# Autodesk Inventor assembly: SaponseEx
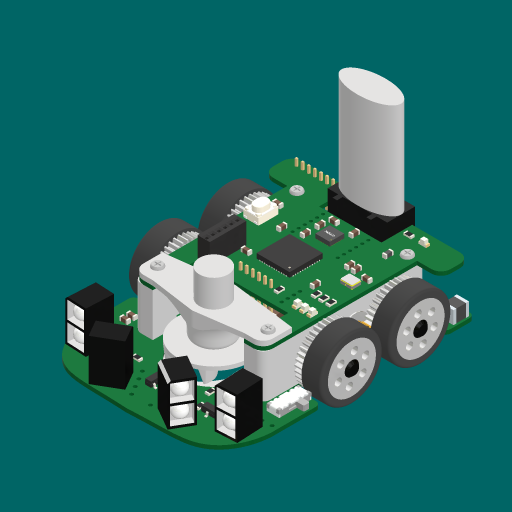
[picture p0: Inventor's stored thumbnail of the model, 512x512]
Saved by Autodesk Inventor 2023 (Build 270158000, 158)
## iProperties
Created: 2022-09-02
Part Number: SaponseEx
Document SubType Name: Assembly
Designer: neko2
Mass: 18.3356 g
Surface Area: 212.041 cm^2
Volume: 11.0257 cm^3
Density: 1.66299 g/cm^3
Author: neko2
## Documents named in this file (13)
- C:\Users\hide\Desktop\SaponseEx\CAD\SaponseEx.iam
- C:\Users\hide\Desktop\SaponseEx\CAD\足回り.iam
- C:\Users\hide\Desktop\SaponseEx\CAD\PCB\SaponseEx_PCB.ipt
- C:\Users\hide\Desktop\SaponseEx\CAD\Board_Parts\SNZS-M1_6-4.ipt
- C:\Users\hide\Desktop\SaponseEx\CAD\PCB\Brains_PCB.ipt
- C:\Users\hide\Desktop\SaponseEx\CAD\PCB\EncL_PCB.ipt
- C:\Users\hide\Desktop\SaponseEx\CAD\PCB\EncR_PCB.ipt
- C:\Users\hide\Desktop\SaponseEx\CAD\Board_Parts\Lipo.ipt
- C:\Users\hide\Desktop\SaponseEx\CAD\吸引\FanMotorMount.ipt
- C:\Users\hide\Desktop\SaponseEx\CAD\mirror\足回り_MIR.iam
- C:\Users\hide\Desktop\SaponseEx\CAD\Skirt.ipt
- C:\Users\hide\Desktop\SaponseEx\CAD\吸引\FanMotor.ipt
- C:\Users\hide\Desktop\SaponseEx\CAD\吸引\Fan4.ipt
## Components (19 placed, 12 different names)
1. SaponseEx_PCB:1 — フラッシュ:1, フラッシュ:2, メイト:1, メイト:10, メイト:11, メイト:12, メイト:19, メイト:20, メイト:22, 円柱状:17, メイト:23
2. Lipo:1 — メイト:10, メイト:11, メイト:12
3. Brains_PCB:1 — リジッド:10, リジッド:11, メイト:15, メイト:17, メイト:18, フラッシュ:4, 円柱状:8, メイト:21
4. SNZS-M1_6-4:5 — リジッド:10, 円柱状:13
5. SNZS-M1_6-4:6 — リジッド:11, 円柱状:10
6. SNZS-M1_6-4:7 — リジッド:8, 円柱状:8, 円柱状:9
7. SNZS-M1_6-4:8 — リジッド:9, 円柱状:16
8. SNZS-M1_6-4:2 — リジッド:3, 円柱状:14
9. SNZS-M1_6-4:1 — 円柱状:15, リジッド:12, 円柱状:17
10. SNZS-M1_6-4:4 — リジッド:5, 円柱状:12
11. SNZS-M1_6-4:3 — リジッド:4, 円柱状:11
12. Skirt:1 — リジッド:12, メイト:23, リジッド:5, リジッド:3, リジッド:4
13. FanMotorMount:1 — リジッド:8, リジッド:9, メイト:15, リジッド:13, メイト:24
14. FanMotor:1 — リジッド:13, 円柱状:18
15. Fan4:1 — 円柱状:18, メイト:24
16. EncL_PCB:1 — メイト:16, メイト:17, フラッシュ:3, 対称度:1, フラッシュ:4
17. EncR_PCB:1 — メイト:16, メイト:18, フラッシュ:3, 対称度:1
18. 足回り [sub-assembly] — 円柱状:9, 円柱状:10, 円柱状:11, 円柱状:12, メイト:20, メイト:21
19. 足回り_MIR:1 [sub-assembly] — 円柱状:13, 円柱状:14, 円柱状:15, 円柱状:16, メイト:22
## Relationships (39: Mate 14, CylindricalJoint 11, WeldJoint 9, Flush 4, Symmetry 1)
- フラッシュ:1 [Flush]: SaponseEx_PCB:1
- フラッシュ:2 [Flush]: SaponseEx_PCB:1
- メイト:1 [Mate]: SaponseEx_PCB:1
- リジッド:3 [WeldJoint]: SNZS-M1_6-4:2 ↔ Skirt:1
- リジッド:4 [WeldJoint]: SNZS-M1_6-4:3 ↔ Skirt:1
- リジッド:5 [WeldJoint]: SNZS-M1_6-4:4 ↔ Skirt:1
- リジッド:8 [WeldJoint]: SNZS-M1_6-4:7 ↔ FanMotorMount:1
- リジッド:9 [WeldJoint]: SNZS-M1_6-4:8 ↔ FanMotorMount:1
- メイト:10 [Mate]: SaponseEx_PCB:1 ↔ Lipo:1
- メイト:11 [Mate]: SaponseEx_PCB:1 ↔ Lipo:1
- メイト:12 [Mate] (-0.1 mm): SaponseEx_PCB:1 ↔ Lipo:1
- リジッド:10 [WeldJoint]: Brains_PCB:1 ↔ SNZS-M1_6-4:5
- リジッド:11 [WeldJoint]: Brains_PCB:1 ↔ SNZS-M1_6-4:6
- メイト:15 [Mate]: Brains_PCB:1 ↔ FanMotorMount:1
- メイト:16 [Mate] (7 mm): EncL_PCB:1 ↔ EncR_PCB:1
- メイト:17 [Mate]: Brains_PCB:1 ↔ EncL_PCB:1
- メイト:18 [Mate]: Brains_PCB:1 ↔ EncR_PCB:1
- フラッシュ:3 [Flush]: EncL_PCB:1 ↔ EncR_PCB:1
- 対称度:1 [Symmetry]: EncL_PCB:1 ↔ EncR_PCB:1
- メイト:19 [Mate]: SaponseEx_PCB:1
- フラッシュ:4 [Flush] (-0.2 mm): Brains_PCB:1 ↔ EncL_PCB:1
- 円柱状:8 [CylindricalJoint]: Brains_PCB:1 ↔ SNZS-M1_6-4:7
- 円柱状:9 [CylindricalJoint]: SNZS-M1_6-4:7 ↔ 足回り
- 円柱状:10 [CylindricalJoint]: SNZS-M1_6-4:6 ↔ 足回り
- 円柱状:11 [CylindricalJoint]: SNZS-M1_6-4:3 ↔ 足回り
- 円柱状:12 [CylindricalJoint]: SNZS-M1_6-4:4 ↔ 足回り
- メイト:20 [Mate]: SaponseEx_PCB:1 ↔ 足回り
- メイト:21 [Mate]: Brains_PCB:1 ↔ 足回り
- 円柱状:13 [CylindricalJoint]: SNZS-M1_6-4:5 ↔ 足回り_MIR:1
- 円柱状:14 [CylindricalJoint]: SNZS-M1_6-4:2 ↔ 足回り_MIR:1
- 円柱状:15 [CylindricalJoint]: SNZS-M1_6-4:1 ↔ 足回り_MIR:1
- 円柱状:16 [CylindricalJoint]: SNZS-M1_6-4:8 ↔ 足回り_MIR:1
- メイト:22 [Mate]: SaponseEx_PCB:1 ↔ 足回り_MIR:1
- リジッド:12 [WeldJoint]: SNZS-M1_6-4:1 ↔ Skirt:1
- 円柱状:17 [CylindricalJoint]: SaponseEx_PCB:1 ↔ SNZS-M1_6-4:1
- メイト:23 [Mate]: SaponseEx_PCB:1 ↔ Skirt:1
- リジッド:13 [WeldJoint]: FanMotorMount:1 ↔ FanMotor:1
- 円柱状:18 [CylindricalJoint]: FanMotor:1 ↔ Fan4:1
- メイト:24 [Mate] (0.1 mm): FanMotorMount:1 ↔ Fan4:1
